# Autodesk Inventor assembly: camaravision
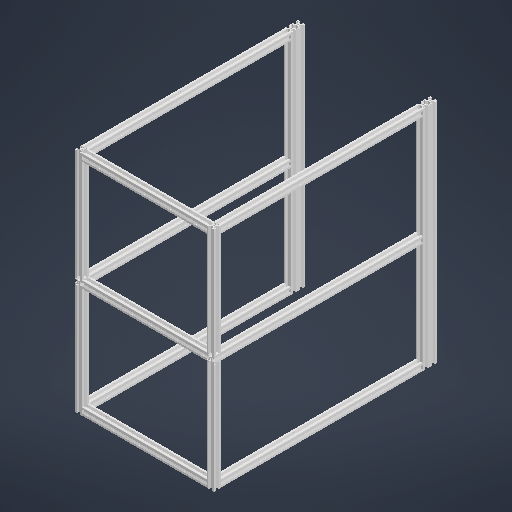
[picture p0: Inventor's stored thumbnail of the model, 512x512]
Saved by Autodesk Inventor 2026.2 (Build 302298010, 298A)
## iProperties
Created: 2026-04-14
Part Number: camaravision
Document SubType Name: Assembly
Designer: grego
Author: grego
## Documents named in this file (6)
- C:\Users\grego\OneDrive\Documentos\PDM\PDM-UVScan\camaravision.iam
- C:\Users\grego\OneDrive\Documentos\PDM\PDM-UVScan\VSLOT20x20x340.ipt
- C:\Users\grego\OneDrive\Documentos\PDM\PDM-UVScan\VSLOT20x20x550.ipt
- C:\Users\grego\OneDrive\Documentos\PDM\PDM-UVScan\VSLOT20x40x620.ipt
- C:\Users\grego\OneDrive\Documentos\PDM\PDM-UVScan\VSLOT20x20x300.ipt
- C:\Users\grego\OneDrive\Documentos\PDM\PDM-UVScan\VSLOT20x20x570.ipt
## Components (15 placed, 5 different names)
1. VSLOT20x20x340:1 — Mate:7, Flush:11, Flush:12, Mate:8, Flush:13, Flush:14
2. VSLOT20x20x550:1 — Mate:1, Flush:1, Flush:2, Mate:2, Flush:3, Flush:4
3. VSLOT20x20x550:3 — Mate:9, Flush:15, Flush:16, Mate:10, Flush:17, Flush:18
4. VSLOT20x40x620:1 — Mate:1, Flush:1, Flush:2, Mate:3
5. VSLOT20x40x620:2 — Mate:10, Flush:17, Flush:18
6. VSLOT20x20x300:1 — Mate:2, Flush:3, Flush:4, Mate:4, Flush:5, Flush:6, Mate:7, Flush:11, Flush:12
7. VSLOT20x20x570:1 — Mate:3, Mate:4, Flush:5, Flush:6, Mate:5, Flush:7, Flush:8, Mate:15, Flush:27, Flush:28
8. VSLOT20x20x300:2 — Mate:5, Flush:7, Flush:8, Mate:6, Flush:9, Flush:10, Mate:14, Flush:25, Flush:26
9. VSLOT20x20x550:4 — Mate:6, Flush:9, Flush:10
10. VSLOT20x20x300:3 — Mate:8, Flush:13, Flush:14, Mate:9, Flush:15, Flush:16, Mate:11, Flush:19, Flush:20
11. VSLOT20x20x570:2 — Mate:11, Flush:19, Flush:20, Mate:12, Flush:21, Flush:22
12. VSLOT20x20x300:4 — Mate:12, Flush:21, Flush:22, Mate:13, Flush:23, Flush:24
13. VSLOT20x20x550:5 — Mate:13, Flush:23, Flush:24
14. VSLOT20x20x340:2 — Mate:14, Flush:25, Flush:26
15. VSLOT20x20x340:3 — Mate:15, Flush:27, Flush:28
## Relationships (43: Flush 28, Mate 15)
- Mate:1: VSLOT20x20x550:1 ↔ VSLOT20x40x620:1
- Flush:1: VSLOT20x20x550:1 ↔ VSLOT20x40x620:1
- Flush:2: VSLOT20x20x550:1 ↔ VSLOT20x40x620:1
- Mate:2: VSLOT20x20x550:1 ↔ VSLOT20x20x300:1
- Flush:3: VSLOT20x20x550:1 ↔ VSLOT20x20x300:1
- Flush:4: VSLOT20x20x550:1 ↔ VSLOT20x20x300:1
- Mate:3: VSLOT20x40x620:1 ↔ VSLOT20x20x570:1
- Mate:4: VSLOT20x20x300:1 ↔ VSLOT20x20x570:1
- Flush:5: VSLOT20x20x300:1 ↔ VSLOT20x20x570:1
- Flush:6: VSLOT20x20x300:1 ↔ VSLOT20x20x570:1
- Mate:5: VSLOT20x20x570:1 ↔ VSLOT20x20x300:2
- Flush:7: VSLOT20x20x570:1 ↔ VSLOT20x20x300:2
- Flush:8: VSLOT20x20x570:1 ↔ VSLOT20x20x300:2
- Mate:6: VSLOT20x20x300:2 ↔ VSLOT20x20x550:4
- Flush:9: VSLOT20x20x300:2 ↔ VSLOT20x20x550:4
- Flush:10: VSLOT20x20x300:2 ↔ VSLOT20x20x550:4
- Mate:7: VSLOT20x20x340:1 ↔ VSLOT20x20x300:1
- Flush:11: VSLOT20x20x340:1 ↔ VSLOT20x20x300:1
- Flush:12: VSLOT20x20x340:1 ↔ VSLOT20x20x300:1
- Mate:8: VSLOT20x20x340:1 ↔ VSLOT20x20x300:3
- Flush:13: VSLOT20x20x340:1 ↔ VSLOT20x20x300:3
- Flush:14: VSLOT20x20x340:1 ↔ VSLOT20x20x300:3
- Mate:9: VSLOT20x20x550:3 ↔ VSLOT20x20x300:3
- Flush:15: VSLOT20x20x550:3 ↔ VSLOT20x20x300:3
- Flush:16: VSLOT20x20x550:3 ↔ VSLOT20x20x300:3
- Mate:10: VSLOT20x20x550:3 ↔ VSLOT20x40x620:2
- Flush:17: VSLOT20x20x550:3 ↔ VSLOT20x40x620:2
- Flush:18: VSLOT20x20x550:3 ↔ VSLOT20x40x620:2
- Mate:11: VSLOT20x20x300:3 ↔ VSLOT20x20x570:2
- Flush:19: VSLOT20x20x300:3 ↔ VSLOT20x20x570:2
- Flush:20: VSLOT20x20x300:3 ↔ VSLOT20x20x570:2
- Mate:12: VSLOT20x20x570:2 ↔ VSLOT20x20x300:4
- Flush:21: VSLOT20x20x570:2 ↔ VSLOT20x20x300:4
- Flush:22: VSLOT20x20x570:2 ↔ VSLOT20x20x300:4
- Mate:13: VSLOT20x20x300:4 ↔ VSLOT20x20x550:5
- Flush:23: VSLOT20x20x300:4 ↔ VSLOT20x20x550:5
- Flush:24: VSLOT20x20x300:4 ↔ VSLOT20x20x550:5
- Mate:14: VSLOT20x20x300:2 ↔ VSLOT20x20x340:2
- Flush:25: VSLOT20x20x300:2 ↔ VSLOT20x20x340:2
- Flush:26: VSLOT20x20x300:2 ↔ VSLOT20x20x340:2
- Mate:15: VSLOT20x20x570:1 ↔ VSLOT20x20x340:3
- Flush:27: VSLOT20x20x570:1 ↔ VSLOT20x20x340:3
- Flush:28: VSLOT20x20x570:1 ↔ VSLOT20x20x340:3
